# Autodesk Inventor assembly: Assembly24
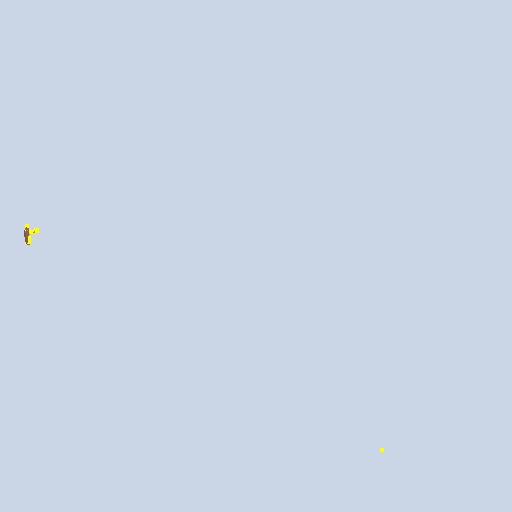
[picture p0: Inventor's stored thumbnail of the model, 512x512]
Saved by Autodesk Inventor 2024.1 (Build 281209000, 209)
## iProperties
Created: 2023-11-10
Part Number: Assembly24
Document SubType Name: Assembly
Designer: luvag
Author: luvag
## Documents named in this file (3)
- C:\Users\luvag\Desktop\Assembly24.iam
- C:\Users\luvag\Desktop\Assembly22.iam
- C:\Users\luvag\Desktop\Oar.ipt
## Components (2 placed, 2 different names)
1. Assembly22:1 [sub-assembly]
2. Oar:1
## Relationships (1: Mate 1)
- [Mate]: Assembly22:1 ↔ Oar:1
